# Autodesk Inventor assembly: mechanical assembly
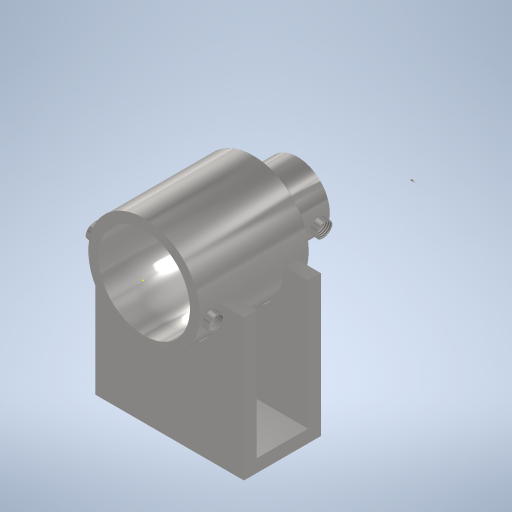
[picture p0: Inventor's stored thumbnail of the model, 512x512]
Saved by Autodesk Inventor 2023 (Build 270158000, 158)
## iProperties
Created: 2022-09-30
Part Number: mechanical assembly
Document SubType Name: Assembly
Designer: station
Author: station
## Documents named in this file (3)
- C:\Users\station\Documents\Project\Liquid-engine-cooling-system\design files\Ethanol engine 5 -inventor files\mechanical assembly.iam
- C:\Users\station\Documents\Project\Liquid-engine-cooling-system\design files\Ethanol engine 5 -inventor files\Support.ipt
- C:\Users\station\Documents\Project\Liquid-engine-cooling-system\design files\Ethanol engine 5 -inventor files\engine basic assembly.iam
## Components (2 placed, 2 different names)
1. Support:1 — Mate:1, Flush:1
2. engine basic assembly:1 [sub-assembly] — Mate:1, Flush:1
## Relationships (2: Mate 1, Flush 1)
- Mate:1: Support:1 ↔ engine basic assembly:1
- Flush:1 (20 mm): Support:1 ↔ engine basic assembly:1
